# Autodesk Inventor assembly: Cylinder_Assembly
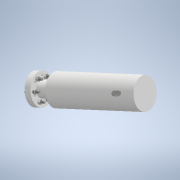
[picture p0: Inventor's stored thumbnail of the model, 180x180]
Saved by Autodesk Inventor 2022 (Build 260153000, 153)
## iProperties
Created: 2022-03-14
Part Number: Cylinder_Assembly
Document SubType Name: Assembly
Designer: karee
Author: karee
## Documents named in this file (6)
- C:\Users\karee\OneDrive\Desktop\Cylinder_Assembly.iam
- C:\Users\karee\OneDrive\Desktop\again.ipt
- C:\Users\karee\OneDrive\Desktop\capp.ipt
- C:\Users\karee\OneDrive\Documents\Inventor\Content Center Files\R2022\en-US\JIS B 1189\JIS B 1189 - M8 x 1.25 - 40.ipt
- C:\Users\karee\OneDrive\Documents\Inventor\Content Center Files\R2022\en-US\ANSI B18.2.4.2M\ANSI B18.2.4.2M - M8x1.25 - 13.ipt
- C:\Users\karee\OneDrive\Documents\Inventor\Content Center Files\R2022\en-US\Parker A(26)\Parker A-Lok Male Taper Thread - Fractional Tube 1_4 x 1_4 (1).ipt
## Components (18 placed, 5 different names)
1. again:1 — Mate:1, Mate:2, Mate:4, Mate:6, Mate:10, Mate:12, Mate:19, Mate:23
2. capp:1 — Mate:1, Mate:2, Insert:2, Insert:3, Insert:4, Insert:5, Insert:6, Insert:7, Mate:17, Mate:18, Mate:21
3. JIS B 1189 - Metric M8 x 40:1 — Insert:2, Mate:20, Mate:22
4. JIS B 1189 - Metric M8 x 40:2 — Insert:3, Mate:9
5. JIS B 1189 - Metric M8 x 40:3 — Insert:4, Mate:3
6. JIS B 1189 - Metric M8 x 40:4 — Insert:5, Mate:13, Mate:15
7. JIS B 1189 - Metric M8 x 40:5 — Insert:6, Mate:11
8. JIS B 1189 - Metric M8 x 40:6 — Insert:7, Mate:5
9. ANSI B18.2.4.2M M8x1.25:1 — Mate:3, Mate:4
10. ANSI B18.2.4.2M M8x1.25:2 — Mate:5, Mate:6
11. ANSI B18.2.4.2M M8x1.25:4 — Mate:9, Mate:10, Mate:14
12. ANSI B18.2.4.2M M8x1.25:5 — Mate:11, Mate:12
13. ANSI B18.2.4.2M M8x1.25:6 — Mate:13, Mate:14, Mate:16
14. ANSI B18.2.4.2M M8x1.25:7 — Mate:15, Mate:16
15. Parker A-Lok Male Taper Thread - Fractional Tube 1/4 x 1/4:1 — Mate:17, Mate:18
16. Parker A-Lok Male Taper Thread - Fractional Tube 1/4 x 1/4:2 — Mate:19
17. ANSI B18.2.4.2M M8x1.25:8 — Mate:20, Mate:21
18. ANSI B18.2.4.2M M8x1.25:9 — Mate:22, Mate:23
## Relationships (27: Mate 21, Insert 6)
- Mate:1: again:1 ↔ capp:1
- Mate:2: again:1 ↔ capp:1
- Insert:2: capp:1 ↔ JIS B 1189 - Metric M8 x 40:1
- Insert:3: capp:1 ↔ JIS B 1189 - Metric M8 x 40:2
- Insert:4: capp:1 ↔ JIS B 1189 - Metric M8 x 40:3
- Insert:5: capp:1 ↔ JIS B 1189 - Metric M8 x 40:4
- Insert:6: capp:1 ↔ JIS B 1189 - Metric M8 x 40:5
- Insert:7: capp:1 ↔ JIS B 1189 - Metric M8 x 40:6
- Mate:3: JIS B 1189 - Metric M8 x 40:3 ↔ ANSI B18.2.4.2M M8x1.25:1
- Mate:4: again:1 ↔ ANSI B18.2.4.2M M8x1.25:1
- Mate:5: JIS B 1189 - Metric M8 x 40:6 ↔ ANSI B18.2.4.2M M8x1.25:2
- Mate:6: again:1 ↔ ANSI B18.2.4.2M M8x1.25:2
- Mate:9: JIS B 1189 - Metric M8 x 40:2 ↔ ANSI B18.2.4.2M M8x1.25:4
- Mate:10: again:1 ↔ ANSI B18.2.4.2M M8x1.25:4
- Mate:11: JIS B 1189 - Metric M8 x 40:5 ↔ ANSI B18.2.4.2M M8x1.25:5
- Mate:12: again:1 ↔ ANSI B18.2.4.2M M8x1.25:5
- Mate:13: JIS B 1189 - Metric M8 x 40:4 ↔ ANSI B18.2.4.2M M8x1.25:6
- Mate:14: ANSI B18.2.4.2M M8x1.25:4 ↔ ANSI B18.2.4.2M M8x1.25:6
- Mate:15: JIS B 1189 - Metric M8 x 40:4 ↔ ANSI B18.2.4.2M M8x1.25:7
- Mate:16: ANSI B18.2.4.2M M8x1.25:6 ↔ ANSI B18.2.4.2M M8x1.25:7
- Mate:17: capp:1 ↔ Parker A-Lok Male Taper Thread - Fractional Tube 1/4 x 1/4:1
- Mate:18: capp:1 ↔ Parker A-Lok Male Taper Thread - Fractional Tube 1/4 x 1/4:1
- Mate:19: again:1 ↔ Parker A-Lok Male Taper Thread - Fractional Tube 1/4 x 1/4:2
- Mate:20: JIS B 1189 - Metric M8 x 40:1 ↔ ANSI B18.2.4.2M M8x1.25:8
- Mate:21: capp:1 ↔ ANSI B18.2.4.2M M8x1.25:8
- Mate:22: JIS B 1189 - Metric M8 x 40:1 ↔ ANSI B18.2.4.2M M8x1.25:9
- Mate:23: again:1 ↔ ANSI B18.2.4.2M M8x1.25:9
